# Autodesk Inventor assembly: PCB
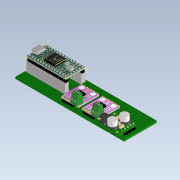
[picture p0: Inventor's stored thumbnail of the model, 180x180]
Saved by Autodesk Inventor 2020 (Build 240168000, 168)
## iProperties
Created: 2021-03-31
Part Number: PCB
Document SubType Name: Assembly
Designer: DELL
Author: DELL
## Documents named in this file (6)
- F:\SoftRobot2.0\FlexipodHardware2.0\FlexipodHardware\Flexipod2.0\PCB\PCB2.0\PCB.iam
- F:\SoftRobot2.0\FlexipodHardware2.0\FlexipodHardware\Flexipod2.0\PCB\teensy_4.0\teensy_4.0.iam
- F:\SoftRobot2.0\FlexipodHardware2.0\FlexipodHardware\Flexipod2.0\PCB\CAN_transceiver\CAN_transceiver_with_pins.iam
- F:\SoftRobot2.0\FlexipodHardware2.0\FlexipodHardware\Flexipod2.0\PCB\Voltage_Regulator\d24v50f5-step-down-voltage-regulator.ipt
- F:\SoftRobot2.0\FlexipodHardware2.0\FlexipodHardware\Flexipod2.0\PCB\pins.ipt
- F:\SoftRobot2.0\FlexipodHardware2.0\FlexipodHardware\Flexipod2.0\PCB\PCB2.0\PCB2.0.iam
## Components (9 placed, 5 different names)
1. teensy_4.0:1 [sub-assembly] — Flush:10, Mate:15
2. CAN_transceiver_with_pins:1 [sub-assembly] — Mate:16, Mate:17, Mate:23
3. CAN_transceiver_with_pins:2 [sub-assembly] — Mate:18, Mate:19, Mate:24
4. d24v50f5-step-down-voltage-regulator:1
5. pins:1 — Mate:21
6. pins:2
7. pins:3
8. pins:4 — Mate:20, Mate:22
9. PCB2.0:1 [sub-assembly] — Mate:14, Flush:8, Flush:9, Flush:10, Mate:15, Mate:16, Mate:17, Mate:18, Mate:19, Mate:20, Mate:21, Mate:22, Mate:23, Mate:24
## Relationships (26: Mate 17, Flush 9)
- [Flush]: pins:1 ↔ pins:2
- [Flush]: pins:2 ↔ pins:3
- [Flush]: pins:3 ↔ pins:4
- [Flush]: pins:1 ↔ pins:2
- [Flush]: pins:2 ↔ pins:3
- [Flush]: pins:3 ↔ pins:4
- [Mate]: pins:3 ↔ pins:4
- [Mate]: pins:2 ↔ pins:3
- [Mate]: pins:1 ↔ pins:2
- [Mate]: d24v50f5-step-down-voltage-regulator:1 ↔ pins:1
- [Mate]: d24v50f5-step-down-voltage-regulator:1 ↔ pins:1
- [Mate]: d24v50f5-step-down-voltage-regulator:1 ↔ pins:4
- Mate:14: PCB2.0:1
- Flush:8: PCB2.0:1
- Flush:9: PCB2.0:1
- Flush:10: teensy_4.0:1 ↔ PCB2.0:1
- Mate:15: teensy_4.0:1 ↔ PCB2.0:1
- Mate:16: CAN_transceiver_with_pins:1 ↔ PCB2.0:1
- Mate:17: CAN_transceiver_with_pins:1 ↔ PCB2.0:1
- Mate:18: CAN_transceiver_with_pins:2 ↔ PCB2.0:1
- Mate:19: CAN_transceiver_with_pins:2 ↔ PCB2.0:1
- Mate:20: pins:4 ↔ PCB2.0:1
- Mate:21: pins:1 ↔ PCB2.0:1
- Mate:22: pins:4 ↔ PCB2.0:1
- Mate:23: CAN_transceiver_with_pins:1 ↔ PCB2.0:1
- Mate:24: CAN_transceiver_with_pins:2 ↔ PCB2.0:1
## Named parameters: d18_d13 = 0 mm, d19_d14 = 0 mm, d20_d15 = 0 mm, d21_d16 = 0 mm
